# Autodesk Inventor assembly: CrankAssem
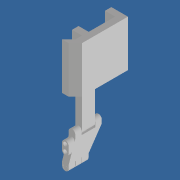
[picture p0: Inventor's stored thumbnail of the model, 180x180]
Saved by Autodesk Inventor 2020 (Build 240168000, 168)
## iProperties
Created: 2019-12-22
Part Number: CrankAssem
Document SubType Name: Assembly
Designer: Jack
Author: Jack
## Documents named in this file (4)
- D:\Code\Python\EV3_Cuber\3D Model\CrankAssem.iam
- D:\Code\Python\EV3_Cuber\3D Model\MotorHolder_X_R.ipt
- D:\Code\Python\EV3_Cuber\3D Model\Crank0.ipt
- D:\Code\Python\EV3_Cuber\3D Model\Crank1.ipt
## Components (3 placed, 3 different names)
1. MotorHolder_X_R:1 — Rotational:1
2. Crank0:1 — Rotational:2
3. Crank1:1 — Rotational:1, Rotational:2
## Relationships (2: RevoluteJoint 2)
- Rotational:1 [RevoluteJoint]: MotorHolder_X_R:1 ↔ Crank1:1
- Rotational:2 [RevoluteJoint]: Crank0:1 ↔ Crank1:1
